# Autodesk Inventor assembly: catapfc3
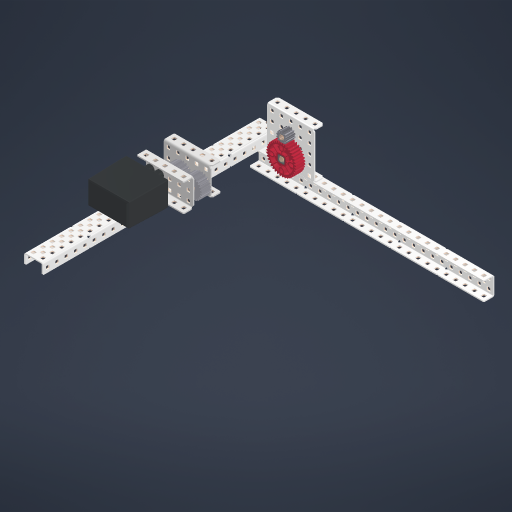
[picture p0: Inventor's stored thumbnail of the model, 512x512]
Saved by Autodesk Inventor 2024 (Build 280153000, 153)
## iProperties
Created: 2023-10-21
Part Number: catapfc3
Document SubType Name: Assembly
Designer: macbook
Author: macbook
## Documents named in this file (9)
- \\Mac\Home\Desktop\code\1599V-VRC\Cad\Assembly\v2\catapfc3.iam
- \\Mac\Home\Desktop\code\1599V-VRC\Cad\Structure\C Channel\Aluminum 1x2x1\Alu C 1x2x1x25.ipt
- \\Mac\Home\Desktop\code\1599V-VRC\Cad\Motion\Gears\HS Gear\HS 12T Gear, No Insert.iam
- \\Mac\Home\Desktop\code\1599V-VRC\Cad\Motion\Gears\HS Gear.iam
- \\Mac\Home\Desktop\code\1599V-VRC\Cad\Motion\Gears\HS Gear\HS 24T Gear, No Insert.iam
- \\Mac\Home\Desktop\code\1599V-VRC\Cad\Motion\Gears\HS Gear\HS 36T Gear, No Insert.iam
- \\Mac\Home\Desktop\code\1599V-VRC\Cad\Electronics\V5 Simple Motor.ipt
- \\Mac\Home\Desktop\code\1599V-VRC\Cad\Structure\C Channel\old\Aluminum 1x5x1\Alu C 1x5x1x5.ipt
- \\Mac\Home\Desktop\code\1599V-VRC\Cad\Structure\C Channel\Aluminum 1x3x1\Alu C 1x3x1x5.ipt
## Components (10 placed, 7 different names)
1. Alu C 1x2x1x25:1 — Insert:9, Insert:10
2. Alu C 1x2x1x25:2 — Insert:13, Insert:14, Insert:15, Insert:16
3. HS 12T Gear, No Insert:1 [sub-assembly] — Insert:11
4. HS 24T Gear, No Insert:2 [sub-assembly]
5. HS 24T Gear, No Insert:4 [sub-assembly]
6. HS 36T Gear, No Insert:6 [sub-assembly] — Insert:12
7. V5 Simple Motor:2
8. Alu C 1x5x1x5:1 — Insert:9, Insert:10, Insert:11, Insert:12
9. Alu C 1x3x1x5:1 — Insert:15, Insert:16
10. Alu C 1x3x1x5:2 — Insert:13, Insert:14
## Relationships (10: Insert 10)
- [Insert] (25.4 mm): Alu C 1x2x1x25:1 ↔ Alu C 1x2x1x25:2
- [Insert] (25.4 mm): Alu C 1x2x1x25:1 ↔ Alu C 1x2x1x25:2
- Insert:9: Alu C 1x2x1x25:1 ↔ Alu C 1x5x1x5:1
- Insert:10: Alu C 1x2x1x25:1 ↔ Alu C 1x5x1x5:1
- Insert:11: HS 12T Gear, No Insert:1 ↔ Alu C 1x5x1x5:1
- Insert:12: HS 36T Gear, No Insert:6 ↔ Alu C 1x5x1x5:1
- Insert:13: Alu C 1x2x1x25:2 ↔ Alu C 1x3x1x5:2
- Insert:14: Alu C 1x2x1x25:2 ↔ Alu C 1x3x1x5:2
- Insert:15: Alu C 1x2x1x25:2 ↔ Alu C 1x3x1x5:1
- Insert:16: Alu C 1x2x1x25:2 ↔ Alu C 1x3x1x5:1
